# Autodesk Inventor assembly: openmv4_h7
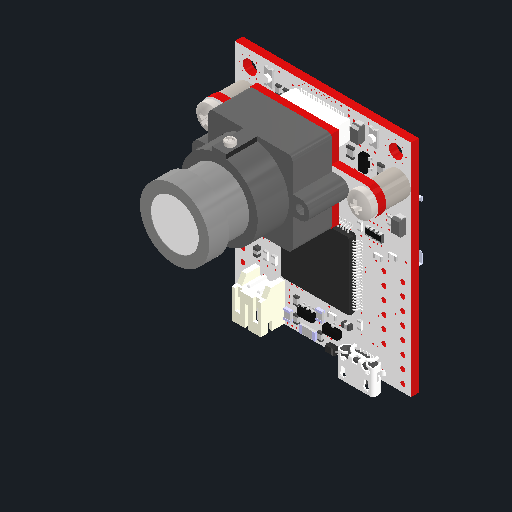
[picture p0: Inventor's stored thumbnail of the model, 512x512]
Saved by Autodesk Inventor 2023.2 (Build 272271030, 271C)
## iProperties
Created: 2019-09-24
Part Number: openmv4_h7
Description: STEP AP214
Document SubType Name: Assembly
Designer: Elias Braun
Sending System: SolidWorks 2016
Preprocessor: SwSTEP 2.0
Title: openmv4_h7.STEP
Revision Number: ANY
## Documents named in this file (9)
- C:\Users\Elias Braun\Nextcloud2\RoboCup2023\Cam\OpenMV H7\OpenMVH7openmv4_h7.iam
- C:\Users\Elias Braun\Nextcloud2\RoboCup2023\Cam\OpenMV H7\OpenMVH7openmv4_h7_base.iam
- C:\Users\Elias Braun\Nextcloud2\RoboCup2023\Cam\OpenMV H7\OpenMVH7openmv4_ov7725.iam
- C:\Users\Elias Braun\Nextcloud2\RoboCup2023\Cam\OpenMV H7\OpenMVH7pan head cross recess screw_iso_ISO 7045 - M2.5 x 5 - Z - 5N.ipt
- C:\Users\Elias Braun\Nextcloud2\RoboCup2023\Cam\OpenMV H7\OpenMVH7microsd card.ipt
- C:\Users\Elias Braun\Nextcloud2\RoboCup2023\Cam\OpenMV H7\OpenMVH7LENS_Standard.ipt
- C:\Users\Elias Braun\Nextcloud2\RoboCup2023\Cam\OpenMV H7\OpenMVH7LENS_Wide.ipt
- C:\Users\Elias Braun\Nextcloud2\RoboCup2023\Cam\OpenMV H7\OpenMVH7Micro USB connector.ipt
- C:\Users\Elias Braun\Nextcloud2\RoboCup2023\Cam\OpenMV H7\OpenMVH7pan head cross recess screw_iso_ISO 7045 - M1 x 4 - Z - 4S.ipt
## Components (9 placed, 9 different names)
1. openmv4_h7_base_® ã¬®«ç ­¨î_1 [sub-assembly] — Mate:3, Mate:4, Mate:5, Mate:6, Mate:7
2. openmv4_ov7725_® ã¬®«ç ­¨î_2 [sub-assembly] — Mate:1, Mate:2, Mate:3, Mate:4, Mate:5, Mate:8, Mate:9, Mate:10, Mate:11, Mate:13
3. pan head cross recess screw_iso_ISO 7045 - M2.5 x 5 - Z - 5N_3 — Mate:7, Mate:8
4. pan head cross recess screw_iso_ISO 7045 - M2.5 x 5 - Z - 5N_4 — Mate:6, Mate:9
5. microsd card_5
6. LENS_Standard_® ã¬®«ç ­¨î_6 — Mate:10, Mate:11, Mate:12
7. LENS_Wide_® ã¬®«ç ­¨î_7 — Mate:12, Mate:13
8. Micro USB connector_8
9. pan head cross recess screw_iso_ISO 7045 - M1 x 4 - Z - 4S_9 — Mate:1, Mate:2
## Relationships (13: Mate 13)
- Mate:1: openmv4_ov7725_® ã¬®«ç ­¨î_2 ↔ pan head cross recess screw_iso_ISO 7045 - M1 x 4 - Z - 4S_9
- Mate:2: openmv4_ov7725_® ã¬®«ç ­¨î_2 ↔ pan head cross recess screw_iso_ISO 7045 - M1 x 4 - Z - 4S_9
- Mate:3: openmv4_h7_base_® ã¬®«ç ­¨î_1 ↔ openmv4_ov7725_® ã¬®«ç ­¨î_2
- Mate:4: openmv4_h7_base_® ã¬®«ç ­¨î_1 ↔ openmv4_ov7725_® ã¬®«ç ­¨î_2
- Mate:5: openmv4_h7_base_® ã¬®«ç ­¨î_1 ↔ openmv4_ov7725_® ã¬®«ç ­¨î_2
- Mate:6: openmv4_h7_base_® ã¬®«ç ­¨î_1 ↔ pan head cross recess screw_iso_ISO 7045 - M2.5 x 5 - Z - 5N_4
- Mate:7: openmv4_h7_base_® ã¬®«ç ­¨î_1 ↔ pan head cross recess screw_iso_ISO 7045 - M2.5 x 5 - Z - 5N_3
- Mate:8: openmv4_ov7725_® ã¬®«ç ­¨î_2 ↔ pan head cross recess screw_iso_ISO 7045 - M2.5 x 5 - Z - 5N_3
- Mate:9: openmv4_ov7725_® ã¬®«ç ­¨î_2 ↔ pan head cross recess screw_iso_ISO 7045 - M2.5 x 5 - Z - 5N_4
- Mate:10: openmv4_ov7725_® ã¬®«ç ­¨î_2 ↔ LENS_Standard_® ã¬®«ç ­¨î_6
- Mate:11 (5 mm): openmv4_ov7725_® ã¬®«ç ­¨î_2 ↔ LENS_Standard_® ã¬®«ç ­¨î_6
- Mate:12: LENS_Standard_® ã¬®«ç ­¨î_6 ↔ LENS_Wide_® ã¬®«ç ­¨î_7
- Mate:13 (10 mm): openmv4_ov7725_® ã¬®«ç ­¨î_2 ↔ LENS_Wide_® ã¬®«ç ­¨î_7
